# Autodesk Inventor assembly: Engine - Blank Slate
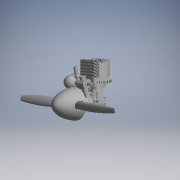
[picture p0: Inventor's stored thumbnail of the model, 180x180]
Saved by Autodesk Inventor 2016 (Build 200138000, 138)
## iProperties
Created: 2012-08-14
Part Number: Engine - Blank Slate
Document SubType Name: Assembly
Designer: John
Author: John
## Documents named in this file (37)
- C:\Users\John Helfen\Desktop\Exercise Files\15_Assembly visualization techniques\15_01\Engine - Blank Slate.iam
- C:\Users\John Helfen\Desktop\Exercise Files\15_Assembly visualization techniques\15_01\Engine Block.ipt
- C:\Users\John Helfen\Desktop\Exercise Files\15_Assembly visualization techniques\15_01\Crankshaft.ipt
- C:\Users\John Helfen\Desktop\Exercise Files\15_Assembly visualization techniques\15_01\Pulley Shaft.ipt
- C:\Users\John Helfen\Desktop\Exercise Files\15_Assembly visualization techniques\15_01\Sleeve.ipt
- C:\Users\John Helfen\Desktop\Exercise Files\15_Assembly visualization techniques\15_01\Piston Shaft.ipt
- C:\Users\John Helfen\Desktop\Exercise Files\15_Assembly visualization techniques\15_01\Piston.ipt
- C:\Users\John Helfen\Desktop\Exercise Files\15_Assembly visualization techniques\15_01\Piston Pin.ipt
- C:\Users\John Helfen\Desktop\Exercise Files\15_Assembly visualization techniques\15_01\Crank Arm.ipt
- C:\Users\John Helfen\Desktop\Exercise Files\15_Assembly visualization techniques\15_01\Face Plate.ipt
- C:\Users\John Helfen\Desktop\Exercise Files\15_Assembly visualization techniques\15_01\washer4.ipt
- C:\Users\John Helfen\Desktop\Exercise Files\15_Assembly visualization techniques\15_01\Screw Lock.ipt
- C:\Users\John Helfen\Desktop\Exercise Files\15_Assembly visualization techniques\15_01\Beveled Sleeve.ipt
- C:\Users\John Helfen\Desktop\Exercise Files\15_Assembly visualization techniques\15_01\Clutch Housing.ipt
- C:\Users\John Helfen\Desktop\Exercise Files\15_Assembly visualization techniques\15_01\Brake Pad.ipt
- C:\Users\John Helfen\Desktop\Exercise Files\15_Assembly visualization techniques\15_01\Clutch Sleeve14.ipt
- C:\Users\John Helfen\Desktop\Exercise Files\15_Assembly visualization techniques\15_01\Clutch Bearing.ipt
- C:\Users\John Helfen\Desktop\Exercise Files\15_Assembly visualization techniques\15_01\Clutch Sleeve11.ipt
- C:\Users\John Helfen\Desktop\Exercise Files\15_Assembly visualization techniques\15_01\Carburetor.iam
- C:\Users\John Helfen\Desktop\Exercise Files\15_Assembly visualization techniques\15_01\Heat Sink.ipt
- C:\Users\John Helfen\Desktop\Exercise Files\15_Assembly visualization techniques\15_01\Starter Cover.ipt
- C:\Users\John Helfen\Desktop\Exercise Files\15_Assembly visualization techniques\15_01\Horseshoe Clip.ipt
- C:\Users\John Helfen\Desktop\Exercise Files\15_Assembly visualization techniques\15_01\ANSI B18.3 - 3-48 UNC - 0.375(31).ipt
- C:\Users\John Helfen\Desktop\Exercise Files\15_Assembly visualization techniques\15_01\ANSI B18.3 - 2-56 UNC - 0.375(31).ipt
- C:\Users\John Helfen\Desktop\Exercise Files\15_Assembly visualization techniques\15_01\Muffler.ipt
- C:\Users\John Helfen\Desktop\Exercise Files\15_Assembly visualization techniques\15_01\ANSI B18.3 - 4-40 UNC - 0.875(31).ipt
- C:\Users\John Helfen\Desktop\Exercise Files\15_Assembly visualization techniques\15_01\Muffler Tip.ipt
- C:\Users\John Helfen\Desktop\Exercise Files\15_Assembly visualization techniques\15_01\Starter Handle.ipt
- C:\Users\John Helfen\Desktop\Exercise Files\15_Assembly visualization techniques\15_01\ANSI B18.3 - 1-64 UNC - UNC - 0.25(1).ipt
- C:\Users\John Helfen\Desktop\Exercise Files\15_Assembly visualization techniques\15_01\Clutch Prop Mount.ipt
- C:\Users\John Helfen\Desktop\Exercise Files\15_Assembly visualization techniques\15_01\Prop Mount.ipt
- C:\Users\John Helfen\Desktop\Exercise Files\15_Assembly visualization techniques\15_01\Prop.ipt
- C:\Users\John Helfen\Desktop\Exercise Files\15_Assembly visualization techniques\15_01\Cone.ipt
- C:\Users\John Helfen\Desktop\Exercise Files\15_Assembly visualization techniques\15_01\Crankshaft Cover.ipt
- C:\Users\John Helfen\Desktop\Exercise Files\15_Assembly visualization techniques\15_01\ANSI B18.3 - 10-24 UNC - UNC - 0.5(1).ipt
- C:\Users\John Helfen\Desktop\Exercise Files\15_Assembly visualization techniques\15_01\ANSI B18.2.2 - 1_4 - 20(3).ipt
- C:\Users\John Helfen\Desktop\Exercise Files\15_Assembly visualization techniques\15_01\ASME B18.21.1 - No. 10. Carbon Steel(4).ipt
## Components (50 placed, 36 different names)
1. Engine Block:1 — Mate:1, Mate:2, Insert:1, Mate:8, Insert:2, Mate:16, Mate:21, Flush:1, Mate:42, Angle:1, Mate:43, Mate:47, Mate:49, Mate:50, Mate:51, Insert:11, Insert:12, Mate:57, Mate:58, Mate:59, Flush:3
2. Crankshaft:1 — Mate:1, Mate:2, Mate:3, Mate:4, Mate:11, Mate:13, Mate:23, Mate:24, Mate:25, Angle:6, DRIVE THIS, Mate:69
3. Pulley Shaft:1 — Mate:3, Mate:4, Mate:7, Mate:17, Mate:18, Mate:19
4. Sleeve:1 — Mate:7, Mate:20
5. Piston Shaft:1 — Insert:1, Mate:8, Mate:12, Mate:48
6. Piston:1 — Mate:10, Mate:12, Mate:14, Mate:15
7. Piston Pin:1 — Mate:9, Mate:10, Mate:14, Mate:15
8. Crank Arm:1 — Mate:9, Mate:11, Mate:13
9. Face Plate:1 — Insert:2, Mate:16, Mate:17, Mate:52, Mate:60, Mate:61, Insert:14, Insert:15, Insert:16, Insert:17, DRIVE THIS
10. washer4:1 — Mate:18, Mate:19, Mate:20
11. Screw Lock:1 — Mate:21, Flush:1
12. Beveled Sleeve:1 — Mate:23, Flush:2
13. Clutch Housing:1 — Mate:24, Flush:2, Mate:27, Mate:29, Mate:30, Mate:31, Mate:32, Mate:47
14. Brake Pad:1 — Mate:31, Mate:32, Tangent:2
15. Brake Pad:2 — Mate:29, Mate:30, Tangent:1, Mate:41
16. Clutch Sleeve14:1 — Mate:25, Mate:27, Mate:33, Mate:34, Mate:37, Mate:39, Mate:53, Mate:54
17. Clutch Bearing:1 — Mate:33, Mate:35
18. Clutch Prop Mount:1 — Mate:34, Mate:35, Tangent:1, Tangent:2, Mate:38, Mate:41, Mate:62, Mate:63, Mate:68
19. Clutch Bearing:2 — Mate:37, Mate:38, Mate:40
20. Clutch Sleeve11:1 — Mate:39, Mate:40
21. Carburetor:1 [sub-assembly] — Mate:42, Angle:1, Mate:43
22. Heat Sink:1 — Mate:48, Mate:49, Mate:50, Mate:51, Insert:3, Insert:4, Insert:5, Insert:6
23. Starter Cover:1 — Mate:52, Insert:7, Insert:8, Insert:9, Insert:10, Mate:60, Mate:61, Insert:13
24. Horseshoe Clip:1 — Mate:53, Mate:54
25. Muffler Tip:1 — Mate:55, Angle:2, Mate:56
26. Muffler:1 — Mate:55, Angle:2, Mate:56, Mate:57, Mate:58, Mate:59
27. Starter Handle:1 — Insert:13
28. Hexagon Socket Head Cap Screw - Inch No. 3 - 48 UNC - 3/8:1 — Insert:3
29. Hexagon Socket Head Cap Screw - Inch No. 3 - 48 UNC - 3/8:2 — Insert:4
30. Hexagon Socket Head Cap Screw - Inch No. 3 - 48 UNC - 3/8:3 — Insert:5
31. Hexagon Socket Head Cap Screw - Inch No. 3 - 48 UNC - 3/8:4 — Insert:6
32. Hexagon Socket Head Cap Screw - Inch No. 2 - 56 UNC - 3/8:1 — Insert:7
33. Hexagon Socket Head Cap Screw - Inch No. 2 - 56 UNC - 3/8:2 — Insert:8
34. Hexagon Socket Head Cap Screw - Inch No. 2 - 56 UNC - 3/8:3 — Insert:9
35. Hexagon Socket Head Cap Screw - Inch No. 2 - 56 UNC - 3/8:4 — Insert:10
36. Hexagon Socket Head Cap Screw - Inch No. 4 - 40 UNC - 7/8:1 — Insert:11
37. Hexagon Socket Head Cap Screw - Inch No. 4 - 40 UNC - 7/8:2 — Insert:12
38. Hexagon Socket Button Head Cap Screw - Inch 1 - 64 x 1/4:1 — Insert:14
39. Hexagon Socket Button Head Cap Screw - Inch 1 - 64 x 1/4:2 — Insert:15
40. Hexagon Socket Button Head Cap Screw - Inch 1 - 64 x 1/4:3 — Insert:16
41. Hexagon Socket Button Head Cap Screw - Inch 1 - 64 x 1/4:4 — Insert:17
42. Prop Mount:1 — Mate:62, Mate:63, Mate:64, Mate:65, Mate:66, Mate:67, Angle:4, Insert:20, Insert:21, Insert:22
43. Prop:1 — Mate:64, Mate:65, Angle:4, Mate:68, Angle:5, Angle:6, Insert:23
44. Cone:1 — Mate:66, Mate:67, Angle:5
45. Crankshaft Cover:1 — Flush:3
46. Hexagon Socket Button Head Cap Screw - Inch 10 - 24 x 1/2:1 — Insert:20
47. Hexagon Socket Button Head Cap Screw - Inch 10 - 24 x 1/2:2 — Insert:21
48. Hexagon Socket Button Head Cap Screw - Inch 10 - 24 x 1/2:3 — Insert:22
49. External Tooth Lock Washer - Type A (Inch) No. 10. Carbon Steel:1 — Insert:23, Mate:70
50. Hex Jam Nut - Inch 1/4 - 20:1 — Mate:69, Mate:70
## Relationships (93: Mate 61, Insert 21, Angle 6, Flush 3, Tangent 2)
- Mate:1: Engine Block:1 ↔ Crankshaft:1
- Mate:2: Engine Block:1 ↔ Crankshaft:1
- Mate:3: Crankshaft:1 ↔ Pulley Shaft:1
- Mate:4: Crankshaft:1 ↔ Pulley Shaft:1
- Mate:7: Pulley Shaft:1 ↔ Sleeve:1
- Insert:1: Engine Block:1 ↔ Piston Shaft:1
- Mate:8: Engine Block:1 ↔ Piston Shaft:1
- Mate:9: Piston Pin:1 ↔ Crank Arm:1
- Mate:10: Piston:1 ↔ Piston Pin:1
- Mate:11: Crankshaft:1 ↔ Crank Arm:1
- Mate:12: Piston Shaft:1 ↔ Piston:1
- Mate:13 (0.127 mm): Crankshaft:1 ↔ Crank Arm:1
- Mate:14: Piston:1 ↔ Piston Pin:1
- Mate:15: Piston:1 ↔ Piston Pin:1
- Insert:2: Engine Block:1 ↔ Face Plate:1
- Mate:16: Engine Block:1 ↔ Face Plate:1
- Mate:17: Pulley Shaft:1 ↔ Face Plate:1
- Mate:18: Pulley Shaft:1 ↔ washer4:1
- Mate:19: Pulley Shaft:1 ↔ washer4:1
- Mate:20: Sleeve:1 ↔ washer4:1
- Mate:21: Engine Block:1 ↔ Screw Lock:1
- Flush:1: Engine Block:1 ↔ Screw Lock:1
- Mate:23: Crankshaft:1 ↔ Beveled Sleeve:1
- Mate:24: Crankshaft:1 ↔ Clutch Housing:1
- Flush:2: Beveled Sleeve:1 ↔ Clutch Housing:1
- Mate:25: Crankshaft:1 ↔ Clutch Sleeve14:1
- Mate:27: Clutch Housing:1 ↔ Clutch Sleeve14:1
- Mate:29: Clutch Housing:1 ↔ Brake Pad:2
- Mate:30: Clutch Housing:1 ↔ Brake Pad:2
- Mate:31: Clutch Housing:1 ↔ Brake Pad:1
- Mate:32: Clutch Housing:1 ↔ Brake Pad:1
- Mate:33: Clutch Sleeve14:1 ↔ Clutch Bearing:1
- Mate:34: Clutch Sleeve14:1 ↔ Clutch Prop Mount:1
- Mate:35: Clutch Bearing:1 ↔ Clutch Prop Mount:1
- Tangent:1: Brake Pad:2 ↔ Clutch Prop Mount:1
- Tangent:2: Brake Pad:1 ↔ Clutch Prop Mount:1
- Mate:37: Clutch Sleeve14:1 ↔ Clutch Bearing:2
- Mate:38: Clutch Prop Mount:1 ↔ Clutch Bearing:2
- Mate:39: Clutch Sleeve14:1 ↔ Clutch Sleeve11:1
- Mate:40: Clutch Bearing:2 ↔ Clutch Sleeve11:1
- Mate:41: Brake Pad:2 ↔ Clutch Prop Mount:1
- Mate:42: Engine Block:1 ↔ Carburetor:1
- Angle:1 (0 deg): Engine Block:1 ↔ Carburetor:1
- Mate:43: Engine Block:1 ↔ Carburetor:1
- Mate:47: Engine Block:1 ↔ Clutch Housing:1
- Mate:48: Piston Shaft:1 ↔ Heat Sink:1
- Mate:49: Engine Block:1 ↔ Heat Sink:1
- Mate:50: Engine Block:1 ↔ Heat Sink:1
- Mate:51: Engine Block:1 ↔ Heat Sink:1
- Mate:52: Face Plate:1 ↔ Starter Cover:1
- Mate:53: Clutch Sleeve14:1 ↔ Horseshoe Clip:1
- Mate:54: Clutch Sleeve14:1 ↔ Horseshoe Clip:1
- Mate:55: Muffler Tip:1 ↔ Muffler:1
- Angle:2 (0 deg): Muffler Tip:1 ↔ Muffler:1
- Mate:56: Muffler Tip:1 ↔ Muffler:1
- Mate:57: Engine Block:1 ↔ Muffler:1
- Mate:58: Engine Block:1 ↔ Muffler:1
- Mate:59: Engine Block:1 ↔ Muffler:1
- Mate:60: Face Plate:1 ↔ Starter Cover:1
- Mate:61: Face Plate:1 ↔ Starter Cover:1
- Insert:13: Starter Cover:1 ↔ Starter Handle:1
- Insert:3: Heat Sink:1 ↔ Hexagon Socket Head Cap Screw - Inch No. 3 - 48 UNC - 3/8:1
- Insert:4: Heat Sink:1 ↔ Hexagon Socket Head Cap Screw - Inch No. 3 - 48 UNC - 3/8:2
- Insert:5: Heat Sink:1 ↔ Hexagon Socket Head Cap Screw - Inch No. 3 - 48 UNC - 3/8:3
- Insert:6: Heat Sink:1 ↔ Hexagon Socket Head Cap Screw - Inch No. 3 - 48 UNC - 3/8:4
- Insert:7: Starter Cover:1 ↔ Hexagon Socket Head Cap Screw - Inch No. 2 - 56 UNC - 3/8:1
- Insert:8: Starter Cover:1 ↔ Hexagon Socket Head Cap Screw - Inch No. 2 - 56 UNC - 3/8:2
- Insert:9: Starter Cover:1 ↔ Hexagon Socket Head Cap Screw - Inch No. 2 - 56 UNC - 3/8:3
- Insert:10: Starter Cover:1 ↔ Hexagon Socket Head Cap Screw - Inch No. 2 - 56 UNC - 3/8:4
- Insert:11: Engine Block:1 ↔ Hexagon Socket Head Cap Screw - Inch No. 4 - 40 UNC - 7/8:1
- Insert:12: Engine Block:1 ↔ Hexagon Socket Head Cap Screw - Inch No. 4 - 40 UNC - 7/8:2
- Insert:14: Face Plate:1 ↔ Hexagon Socket Button Head Cap Screw - Inch 1 - 64 x 1/4:1
- Insert:15: Face Plate:1 ↔ Hexagon Socket Button Head Cap Screw - Inch 1 - 64 x 1/4:2
- Insert:16: Face Plate:1 ↔ Hexagon Socket Button Head Cap Screw - Inch 1 - 64 x 1/4:3
- Insert:17: Face Plate:1 ↔ Hexagon Socket Button Head Cap Screw - Inch 1 - 64 x 1/4:4
- Angle:6 (0 deg): Crankshaft:1 ↔ Prop:1
- DRIVE THIS [Angle] (0 deg): Crankshaft:1 ↔ Face Plate:1
- Mate:62: Clutch Prop Mount:1 ↔ Prop Mount:1
- Mate:63: Clutch Prop Mount:1 ↔ Prop Mount:1
- Mate:64: Prop Mount:1 ↔ Prop:1
- Mate:65: Prop Mount:1 ↔ Prop:1
- Mate:66: Prop Mount:1 ↔ Cone:1
- Mate:67: Prop Mount:1 ↔ Cone:1
- Angle:4 (0 deg): Prop Mount:1 ↔ Prop:1
- Mate:68: Clutch Prop Mount:1 ↔ Prop:1
- Angle:5 (0 deg): Prop:1 ↔ Cone:1
- Flush:3: Engine Block:1 ↔ Crankshaft Cover:1
- Insert:20: Prop Mount:1 ↔ Hexagon Socket Button Head Cap Screw - Inch 10 - 24 x 1/2:1
- Insert:21: Prop Mount:1 ↔ Hexagon Socket Button Head Cap Screw - Inch 10 - 24 x 1/2:2
- Insert:22: Prop Mount:1 ↔ Hexagon Socket Button Head Cap Screw - Inch 10 - 24 x 1/2:3
- Insert:23: Prop:1 ↔ External Tooth Lock Washer - Type A (Inch) No. 10. Carbon Steel:1
- Mate:69: Crankshaft:1 ↔ Hex Jam Nut - Inch 1/4 - 20:1
- Mate:70: External Tooth Lock Washer - Type A (Inch) No. 10. Carbon Steel:1 ↔ Hex Jam Nut - Inch 1/4 - 20:1
